# Autodesk Inventor assembly: AssemblyFidget
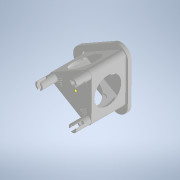
[picture p0: Inventor's stored thumbnail of the model, 180x180]
Saved by Autodesk Inventor 2022.4 (Build 264492010, 492A)
## iProperties
Created: 2023-09-20
Part Number: AssemblyFidget
Document SubType Name: Assembly
Designer: tmass
Author: tmass
## Documents named in this file (5)
- C:\Users\tmass\OneDrive\Bureau\UFO paper\3D models\Fidget\Inventor\AssemblyFidget.iam
- C:\Users\tmass\OneDrive\Bureau\UFO paper\3D models\Fidget\Inventor\Reactor small aircooled.ipt
- C:\Users\tmass\OneDrive\Bureau\UFO paper\3D models\Fidget\Inventor\Lid small.ipt
- C:\Users\tmass\OneDrive\Bureau\UFO paper\3D models\Fidget\Inventor\mini fidget foot.ipt
- C:\Users\tmass\OneDrive\Bureau\UFO paper\3D models\Fidget\Inventor\Coil holder.ipt
## Components (6 placed, 4 different names)
1. Reactor small aircooled:1 — Mate:1, Mate:2, Mate:3, Mate:4, Mate:5, Mate:6, Mate:7, Mate:8, Mate:9, Mate:10, Mate:11, Mate:12
2. Lid small:1 — Mate:4, Mate:5, Mate:6
3. mini fidget foot:1 — Mate:8, Mate:10
4. mini fidget foot:2 — Mate:7, Mate:11
5. mini fidget foot:3 — Mate:9, Mate:12
6. Coil holder:1 — Mate:1, Mate:2, Mate:3
## Relationships (12: Mate 12)
- Mate:1: Reactor small aircooled:1 ↔ Coil holder:1
- Mate:2: Reactor small aircooled:1 ↔ Coil holder:1
- Mate:3 (1 mm): Reactor small aircooled:1 ↔ Coil holder:1
- Mate:4: Reactor small aircooled:1 ↔ Lid small:1
- Mate:5: Reactor small aircooled:1 ↔ Lid small:1
- Mate:6: Reactor small aircooled:1 ↔ Lid small:1
- Mate:7: Reactor small aircooled:1 ↔ mini fidget foot:2
- Mate:8: Reactor small aircooled:1 ↔ mini fidget foot:1
- Mate:9: Reactor small aircooled:1 ↔ mini fidget foot:3
- Mate:10: Reactor small aircooled:1 ↔ mini fidget foot:1
- Mate:11: Reactor small aircooled:1 ↔ mini fidget foot:2
- Mate:12: Reactor small aircooled:1 ↔ mini fidget foot:3
